# Autodesk Inventor assembly: BM-M092CS
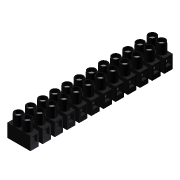
[picture p0: Inventor's stored thumbnail of the model, 180x180]
Saved by Autodesk Inventor 2012 (Build 160160000, 160)
## iProperties
Category: Electrical
Company: Autodesk Inc.
Created: 2008-12-26
Part Number: BM-M092CS
Document SubType Name: Assembly
Designer: Autodesk Inc.
Catalog Web Link: http://web5.automationdirect.com/static/specs/dinmounttb.pdf
Description: Direct Mount Terminal Block
Vendor: AutomationDirect
Author: Autodesk Inc.
## Documents named in this file (3)
- C:\Users\Antonella\Documents\GCC Robotics 2012 - Mechanical\Robot 2.0\Other Models\DirectMountTerminalBlock_AutomationDirect_BM-M092CS.iam
- C:\Users\Antonella\Documents\GCC Robotics 2012 - Mechanical\Robot 2.0\Other Models\DirectMountTerminalBlock_AutomationDirect_BM-M092CS.ipt
- C:\Users\Antonella\Documents\GCC Robotics 2012 - Mechanical\Robot 2.0\Other Models\ISO 1207 - M2.5 x 6.ipt
## Components (25 placed, 2 different names)
1. DirectMountTerminalBlock_AutomationDirect_BM-M092CS:1 — Insert:1
2. ISO 1207 M2.5 x 6:1 — Insert:1
3. ISO 1207 M2.5 x 6:2
4. ISO 1207 M2.5 x 6:3
5. ISO 1207 M2.5 x 6:4
6. ISO 1207 M2.5 x 6:5
7. ISO 1207 M2.5 x 6:6
8. ISO 1207 M2.5 x 6:7
9. ISO 1207 M2.5 x 6:8
10. ISO 1207 M2.5 x 6:9
11. ISO 1207 M2.5 x 6:10
12. ISO 1207 M2.5 x 6:11
13. ISO 1207 M2.5 x 6:12
14. ISO 1207 M2.5 x 6:13
15. ISO 1207 M2.5 x 6:14
16. ISO 1207 M2.5 x 6:15
17. ISO 1207 M2.5 x 6:16
18. ISO 1207 M2.5 x 6:17
19. ISO 1207 M2.5 x 6:18
20. ISO 1207 M2.5 x 6:19
21. ISO 1207 M2.5 x 6:20
22. ISO 1207 M2.5 x 6:21
23. ISO 1207 M2.5 x 6:22
24. ISO 1207 M2.5 x 6:23
25. ISO 1207 M2.5 x 6:24
## Component patterns: (24 elements, first: ISO 1207 M2.5 x 6:1)
## Relationships (1: Insert 1)
- Insert:1: DirectMountTerminalBlock_AutomationDirect_BM-M092CS:1 ↔ ISO 1207 M2.5 x 6:1
